# Autodesk Inventor assembly: Case
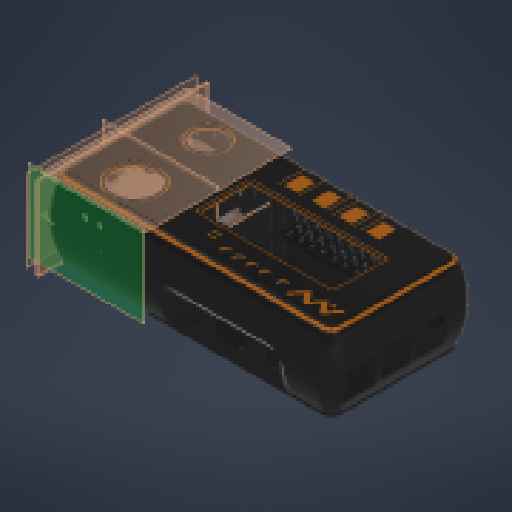
[picture p0: Inventor's stored thumbnail of the model, 512x512]
Saved by Autodesk Inventor 2023 (Build 270158000, 158)
## iProperties
Created: 2022-12-23
Part Number: Case
Document SubType Name: Assembly
Designer: Manuel
Author: Manuel
## Documents named in this file (5)
- C:\workspace\Studium\WST\opcua_netzwerk\Entwicklung Knoten\3D Modell\Case\Case.iam
- C:\workspace\Studium\WST\opcua_netzwerk\Entwicklung Knoten\3D Modell\Case\ComA_Body.ipt
- C:\workspace\Studium\WST\opcua_netzwerk\Entwicklung Knoten\3D Modell\Case\ComA_Dist.ipt
- C:\workspace\Studium\WST\opcua_netzwerk\Entwicklung Knoten\3D Modell\Case\ComB_Body.ipt
- C:\workspace\Studium\WST\opcua_netzwerk\Entwicklung Knoten\3D Modell\Case\ComA_Cover.ipt
## Components (7 placed, 4 different names)
1. ComA_Body:1 — Passend:1, Passend:2, Passend:3, Passend:4, Passend:7, Fluchtend:4, Zylindrisch:1, Passend:8
2. ComA_Dist:1 — Passend:1, Fluchtend:2, Fluchtend:3
3. ComA_Dist:2 — Passend:4, Fluchtend:3, Zylindrisch:1
4. ComA_Dist:3 — Passend:3, Fluchtend:1
5. ComA_Dist:4 — Passend:2, Fluchtend:1, Fluchtend:2
6. ComB_Body:1 — Passend:7, Fluchtend:4
7. ComA_Cover:1 — Passend:8
## Relationships (11: Mate 6, Flush 4, CylindricalJoint 1)
- Passend:1 [Mate]: ComA_Body:1 ↔ ComA_Dist:1
- Passend:2 [Mate]: ComA_Body:1 ↔ ComA_Dist:4
- Passend:3 [Mate]: ComA_Body:1 ↔ ComA_Dist:3
- Passend:4 [Mate]: ComA_Body:1 ↔ ComA_Dist:2
- Fluchtend:1 [Flush]: ComA_Dist:3 ↔ ComA_Dist:4
- Fluchtend:2 [Flush]: ComA_Dist:1 ↔ ComA_Dist:4
- Fluchtend:3 [Flush]: ComA_Dist:1 ↔ ComA_Dist:2
- Passend:7 [Mate]: ComA_Body:1 ↔ ComB_Body:1
- Fluchtend:4 [Flush]: ComA_Body:1 ↔ ComB_Body:1
- Zylindrisch:1 [CylindricalJoint]: ComA_Body:1 ↔ ComA_Dist:2
- Passend:8 [Mate]: ComA_Body:1 ↔ ComA_Cover:1
